# Autodesk Inventor assembly: Shell (1)
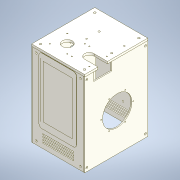
[picture p0: Inventor's stored thumbnail of the model, 180x180]
Saved by Autodesk Inventor 2020 (Build 240168000, 168)
## iProperties
Created: 2020-03-27
Part Number: Shell (1)
Document SubType Name: Assembly
Designer: John K
Author: John K
## Documents named in this file (7)
- C:\GrabCAD\MTL Ventilator Design\Shell (1).iam
- C:\GrabCAD\MTL Ventilator Design\Raspberry Pi 7 Touch Screen LCD v1.ipt
- C:\GrabCAD\MTL Ventilator Design\Component41.ipt
- C:\GrabCAD\MTL Ventilator Design\Component44.ipt
- C:\GrabCAD\MTL Ventilator Design\Component43.ipt
- C:\GrabCAD\MTL Ventilator Design\Component42.ipt
- C:\GrabCAD\MTL Ventilator Design\Component45.ipt
## Components (6 placed, 6 different names)
1. Raspberry Pi 7 Touch Screen LCD v1:1
2. Component41:1 — Flush:1, Mate:1, Mate:2
3. Component44:1 — Mate:2
4. Component43:1
5. Component42:1
6. Component45:1 — Flush:1, Mate:1
## Relationships (3: Mate 2, Flush 1)
- Flush:1: Component41:1 ↔ Component45:1
- Mate:1: Component41:1 ↔ Component45:1
- Mate:2: Component41:1 ↔ Component44:1
